# Autodesk Inventor assembly: 3dacregconv
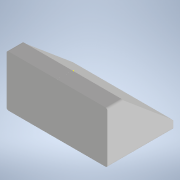
[picture p0: Inventor's stored thumbnail of the model, 180x180]
Saved by Autodesk Inventor 2022 (Build 260153000, 153)
## iProperties
Created: 2022-08-18
Part Number: 3dacregconv
Document SubType Name: Assembly
Designer: HiPeng
Author: HiPeng
## Documents named in this file (5)
- F:\Project\3_phase_firing\3d-cad\3dacregconv.iam
- F:\Project\3_phase_firing\3d-cad\body.ipt
- F:\Project\3_phase_firing\3d-cad\body_MIR.ipt
- F:\Project\3_phase_firing\3d-cad\bottom.ipt
- F:\Project\3_phase_firing\3d-cad\top_cover.ipt
## Components (4 placed, 4 different names)
1. body:1 — Mate:1, Mate:2, Mate:5, Mate:8
2. body_MIR:1 — Mate:3, Mate:4, Mate:6, Mate:7, Mate:9, Mate:10
3. bottom:1 — Flush:1
4. top_cover:1 — Flush:2
## Relationships (12: Mate 10, Flush 2)
- Mate:1: body:1
- Mate:2: body:1
- Mate:3: body_MIR:1
- Mate:4: body_MIR:1
- Mate:5: body:1
- Mate:6: body_MIR:1
- Mate:7: body_MIR:1
- Mate:8: body:1
- Flush:1: bottom:1
- Mate:9: body_MIR:1
- Mate:10: body_MIR:1
- Flush:2: top_cover:1
